# Autodesk Inventor assembly: MainModule
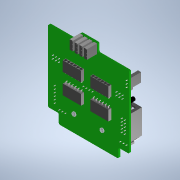
[picture p0: Inventor's stored thumbnail of the model, 180x180]
Saved by Autodesk Inventor 2021 (Build 250183000, 183)
## iProperties
Created: 2021-05-14
Part Number: MainModule
Document SubType Name: Assembly
Designer: ermoz
Author: ermoz
## Documents named in this file (19)
- D:\Moje Wyczyny\My_Poor_Projects\Sneak100_MiniSumo\minisumo-sneak100\mechanics\ElectricElements\MainModule.iam
- D:\Moje Wyczyny\My_Poor_Projects\Sneak100_MiniSumo\minisumo-sneak100\mechanics\ElectricElements\MainBoard.ipt
- D:\Moje Wyczyny\My_Poor_Projects\Sneak100_MiniSumo\minisumo-sneak100\mechanics\ElectricElements\IDC_10_pin_connector.ipt
- D:\Moje Wyczyny\My_Poor_Projects\Sneak100_MiniSumo\minisumo-sneak100\mechanics\ElectricElements\STM32F303RE_LQFP64.ipt
- D:\Moje Wyczyny\My_Poor_Projects\Sneak100_MiniSumo\minisumo-sneak100\mechanics\ElectricElements\SSD1306.ipt
- D:\Moje Wyczyny\My_Poor_Projects\Sneak100_MiniSumo\minisumo-sneak100\mechanics\ElectricElements\TactSwitch_6x6_8mm_SMD.ipt
- D:\Moje Wyczyny\My_Poor_Projects\Sneak100_MiniSumo\minisumo-sneak100\mechanics\ElectricElements\FemaleHeaderPin_1x6.iam
- D:\Moje Wyczyny\My_Poor_Projects\Sneak100_MiniSumo\minisumo-sneak100\mechanics\ElectricElements\Switch_ESP2010_90.ipt
- D:\Moje Wyczyny\My_Poor_Projects\Sneak100_MiniSumo\minisumo-sneak100\mechanics\ElectricElements\S9V11F5.ipt
- D:\Moje Wyczyny\My_Poor_Projects\Sneak100_MiniSumo\minisumo-sneak100\mechanics\ElectricElements\MaleHeaderPin_1x3.iam
- D:\Moje Wyczyny\My_Poor_Projects\Sneak100_MiniSumo\minisumo-sneak100\mechanics\ElectricElements\MaleHeaderPin_1x4.iam
- D:\Moje Wyczyny\My_Poor_Projects\Sneak100_MiniSumo\minisumo-sneak100\mechanics\ElectricElements\TSOP4838.ipt
- D:\Moje Wyczyny\My_Poor_Projects\Sneak100_MiniSumo\minisumo-sneak100\mechanics\ElectricElements\FemaleHeaderPin_1x3.iam
- D:\Moje Wyczyny\My_Poor_Projects\Sneak100_MiniSumo\minisumo-sneak100\mechanics\ElectricElements\FemaleHeaderPin_1x6_90.iam
- D:\Moje Wyczyny\My_Poor_Projects\Sneak100_MiniSumo\minisumo-sneak100\mechanics\PreMadeParts\DistanceRing_4mm.ipt
- D:\Moje Wyczyny\My_Poor_Projects\Sneak100_MiniSumo\minisumo-sneak100\mechanics\PreMadeParts\M2_Short_Bolt.ipt
- D:\Moje Wyczyny\My_Poor_Projects\Sneak100_MiniSumo\minisumo-sneak100\mechanics\ElectricElements\FemaleHeaderPin_2x3_90.iam
- D:\Moje Wyczyny\My_Poor_Projects\Sneak100_MiniSumo\minisumo-sneak100\mechanics\ElectricElements\PinHeaderJumper.ipt
- D:\Moje Wyczyny\My_Poor_Projects\Sneak100_MiniSumo\minisumo-sneak100\mechanics\PreMadeParts\2M_Nut.ipt
## Components (33 placed, 18 different names)
1. MainBoard:1 — Mate:1, Mate:3, Flush:1, Mate:8, Mate:17, Mate:18, Mate:19, Mate:24, Flush:4, Mate:25, Mate:27, Mate:32, Mate:34, Flush:11, Flush:13, Flush:14, Mate:39, Flush:15, Mate:40, Flush:16, Mate:42, Flush:17, Mate:43, Mate:44, Mate:45, Mate:46, Flush:18, Flush:19, Flush:20, Flush:21, Flush:22, Flush:23, Mate:49, Flush:24, Flush:25, Mate:50, Mate:51, Mate:52, Mate:53, Flush:30, Flush:31, Mate:55, Mate:56, Mate:57, Mate:58, Mate:59, Mate:60, Tangent:4, Tangent:5, Tangent:6, Tangent:7, Mate:63, Mate:64, Flush:33, Flush:34, Flush:35
2. IDC_10_pin_connector:1 — Mate:1, Flush:1, Flush:11, Mate:41, Mate:66
3. STM32F303RE_LQFP64:1 — Mate:3
4. SSD1306:1 — Mate:8, Tangent:1, Tangent:2, Tangent:3, Mate:36, Mate:37, Angle:4, Mate:69, Mate:70
5. TactSwitch_6x6_8mm_SMD:1 — Mate:17, Symmetry:1, Flush:2
6. TactSwitch_6x6_8mm_SMD:2 — Mate:18, Mate:20, Angle:3, Flush:2, Flush:3, Mate:35
7. TactSwitch_6x6_8mm_SMD:3 — Mate:19, Symmetry:1, Flush:3, Mate:34, Mate:35, Mate:36
8. FemaleHeaderPin_1x6:1 [sub-assembly] — Mate:24, Flush:13, Flush:14
9. Switch_ESP2010_90:1 — Flush:4, Mate:25, Flush:15
10. S9V11F5:1 — Mate:28, Flush:6, Flush:7
11. MaleHeaderPin_1x3:1 [sub-assembly] — Mate:27, Mate:28, Flush:6, Flush:7
12. MaleHeaderPin_1x4:1 [sub-assembly] — Mate:32, Tangent:1, Tangent:2, Tangent:3
13. TSOP4838:1 — Mate:39
14. TactSwitch_6x6_8mm_SMD:4 — Mate:40, Flush:16, Mate:41
15. MaleHeaderPin_1x3:2 [sub-assembly] — Mate:42, Flush:17, Mate:65, Flush:36, Flush:37, Mate:66
16. FemaleHeaderPin_1x3:1 [sub-assembly] — Mate:43, Flush:18, Flush:23, Mate:48
17. FemaleHeaderPin_1x3:2 [sub-assembly] — Mate:44, Flush:19, Mate:48
18. FemaleHeaderPin_1x3:3 [sub-assembly] — Mate:45, Flush:20, Mate:47
19. FemaleHeaderPin_1x3:4 [sub-assembly] — Mate:46, Flush:21, Flush:22, Mate:47
20. FemaleHeaderPin_1x3:5 [sub-assembly] — Mate:49, Flush:24, Flush:25
21. FemaleHeaderPin_1x6_90:1 [sub-assembly] — Mate:50, Flush:27, Flush:29
22. FemaleHeaderPin_1x6_90:2 [sub-assembly] — Mate:52, Flush:27, Flush:28, Mate:56
23. FemaleHeaderPin_1x6_90:3 [sub-assembly] — Mate:51, Flush:26, Flush:29, Flush:30
24. FemaleHeaderPin_1x6_90:4 [sub-assembly] — Mate:53, Flush:26, Flush:28, Flush:31, Mate:55
25. DistanceRing_4mm:1 — Mate:57, Mate:62
26. DistanceRing_4mm:2 — Mate:58, Mate:61
27. M2_Short_Bolt:1 — Mate:59, Mate:61, Tangent:4, Tangent:6, Mate:67
28. M2_Short_Bolt:2 — Mate:60, Mate:62, Tangent:5, Tangent:7, Mate:68
29. FemaleHeaderPin_2x3_90:1 [sub-assembly] — Mate:63, Flush:32, Flush:33
30. FemaleHeaderPin_2x3_90:2 [sub-assembly] — Mate:64, Flush:32, Flush:34, Flush:35
31. PinHeaderJumper:1 — Mate:65, Flush:36, Flush:37
32. 2M_Nut:1 — Mate:67, Mate:69
33. 2M_Nut:2 — Mate:68, Mate:70
## Relationships (93: Mate 51, Flush 32, Tangent 7, Angle 2, Symmetry 1)
- Mate:1: MainBoard:1 ↔ IDC_10_pin_connector:1
- Mate:3: MainBoard:1 ↔ STM32F303RE_LQFP64:1
- Flush:1: MainBoard:1 ↔ IDC_10_pin_connector:1
- Mate:8 (4 mm): MainBoard:1 ↔ SSD1306:1
- Mate:16
- Mate:17: MainBoard:1 ↔ TactSwitch_6x6_8mm_SMD:1
- Mate:18: MainBoard:1 ↔ TactSwitch_6x6_8mm_SMD:2
- Mate:19: MainBoard:1 ↔ TactSwitch_6x6_8mm_SMD:3
- Mate:20: TactSwitch_6x6_8mm_SMD:2
- Angle:3 (0 deg): TactSwitch_6x6_8mm_SMD:2
- Symmetry:1: TactSwitch_6x6_8mm_SMD:1 ↔ TactSwitch_6x6_8mm_SMD:3
- Mate:21
- Flush:2: TactSwitch_6x6_8mm_SMD:1 ↔ TactSwitch_6x6_8mm_SMD:2
- Flush:3: TactSwitch_6x6_8mm_SMD:2 ↔ TactSwitch_6x6_8mm_SMD:3
- Mate:23
- Mate:24: MainBoard:1 ↔ FemaleHeaderPin_1x6:1
- Flush:4 (1 mm): MainBoard:1 ↔ Switch_ESP2010_90:1
- Mate:25: MainBoard:1 ↔ Switch_ESP2010_90:1
- Mate:27: MainBoard:1 ↔ MaleHeaderPin_1x3:1
- Mate:28: S9V11F5:1 ↔ MaleHeaderPin_1x3:1
- Flush:6: S9V11F5:1 ↔ MaleHeaderPin_1x3:1
- Flush:7: S9V11F5:1 ↔ MaleHeaderPin_1x3:1
- Mate:32: MainBoard:1 ↔ MaleHeaderPin_1x4:1
- Tangent:1 (-0.225 mm): SSD1306:1 ↔ MaleHeaderPin_1x4:1
- Tangent:2 (-0.225 mm): SSD1306:1 ↔ MaleHeaderPin_1x4:1
- Mate:34 (-7 mm): MainBoard:1 ↔ TactSwitch_6x6_8mm_SMD:3
- Tangent:3 (-0.225 mm): SSD1306:1 ↔ MaleHeaderPin_1x4:1
- Mate:35 (7 mm): TactSwitch_6x6_8mm_SMD:2 ↔ TactSwitch_6x6_8mm_SMD:3
- Flush:11 (16 mm): MainBoard:1 ↔ IDC_10_pin_connector:1
- Flush:13 (13 mm): MainBoard:1 ↔ FemaleHeaderPin_1x6:1
- Flush:14 (5 mm): MainBoard:1 ↔ FemaleHeaderPin_1x6:1
- Mate:36 (9.5 mm): SSD1306:1 ↔ TactSwitch_6x6_8mm_SMD:3
- Mate:37: SSD1306:1
- Angle:4 (0 deg): SSD1306:1
- Mate:38
- Mate:39 (3 mm): MainBoard:1 ↔ TSOP4838:1
- Flush:15: MainBoard:1 ↔ Switch_ESP2010_90:1
- Mate:40: MainBoard:1 ↔ TactSwitch_6x6_8mm_SMD:4
- Flush:16 (2.77 mm): MainBoard:1 ↔ TactSwitch_6x6_8mm_SMD:4
- Mate:41 (0.9 mm): IDC_10_pin_connector:1 ↔ TactSwitch_6x6_8mm_SMD:4
- Mate:42: MainBoard:1 ↔ MaleHeaderPin_1x3:2
- Flush:17 (12.5 mm): MainBoard:1 ↔ MaleHeaderPin_1x3:2
- Mate:43: MainBoard:1 ↔ FemaleHeaderPin_1x3:1
- Mate:44: MainBoard:1 ↔ FemaleHeaderPin_1x3:2
- Mate:45: MainBoard:1 ↔ FemaleHeaderPin_1x3:3
- Mate:46: MainBoard:1 ↔ FemaleHeaderPin_1x3:4
- Flush:18 (0.2 mm): MainBoard:1 ↔ FemaleHeaderPin_1x3:1
- Flush:19 (0.4 mm): MainBoard:1 ↔ FemaleHeaderPin_1x3:2
- Flush:20 (0.4 mm): MainBoard:1 ↔ FemaleHeaderPin_1x3:3
- Flush:21 (0.4 mm): MainBoard:1 ↔ FemaleHeaderPin_1x3:4
- Flush:22 (0.4 mm): MainBoard:1 ↔ FemaleHeaderPin_1x3:4
- Flush:23 (0.2 mm): MainBoard:1 ↔ FemaleHeaderPin_1x3:1
- Mate:47 (1.4 mm): FemaleHeaderPin_1x3:3 ↔ FemaleHeaderPin_1x3:4
- Mate:48 (1.5 mm): FemaleHeaderPin_1x3:1 ↔ FemaleHeaderPin_1x3:2
- Mate:49: MainBoard:1 ↔ FemaleHeaderPin_1x3:5
- Flush:24 (0.2 mm): MainBoard:1 ↔ FemaleHeaderPin_1x3:5
- Flush:25 (5.84 mm): MainBoard:1 ↔ FemaleHeaderPin_1x3:5
- Mate:50: MainBoard:1 ↔ FemaleHeaderPin_1x6_90:1
- Mate:51: MainBoard:1 ↔ FemaleHeaderPin_1x6_90:3
- Mate:52: MainBoard:1 ↔ FemaleHeaderPin_1x6_90:2
- Mate:53: MainBoard:1 ↔ FemaleHeaderPin_1x6_90:4
- Flush:26: FemaleHeaderPin_1x6_90:3 ↔ FemaleHeaderPin_1x6_90:4
- Flush:27: FemaleHeaderPin_1x6_90:1 ↔ FemaleHeaderPin_1x6_90:2
- Flush:28: FemaleHeaderPin_1x6_90:2 ↔ FemaleHeaderPin_1x6_90:4
- Flush:29: FemaleHeaderPin_1x6_90:1 ↔ FemaleHeaderPin_1x6_90:3
- Flush:30 (14.92 mm): MainBoard:1 ↔ FemaleHeaderPin_1x6_90:3
- Flush:31 (14.92 mm): MainBoard:1 ↔ FemaleHeaderPin_1x6_90:4
- Mate:55 (-33.74 mm): MainBoard:1 ↔ FemaleHeaderPin_1x6_90:4
- Mate:56 (-32.84 mm): MainBoard:1 ↔ FemaleHeaderPin_1x6_90:2
- Mate:57: MainBoard:1 ↔ DistanceRing_4mm:1
- Mate:58: MainBoard:1 ↔ DistanceRing_4mm:2
- Mate:59: MainBoard:1 ↔ M2_Short_Bolt:1
- Mate:60: MainBoard:1 ↔ M2_Short_Bolt:2
- Mate:61: DistanceRing_4mm:2 ↔ M2_Short_Bolt:1
- Mate:62: DistanceRing_4mm:1 ↔ M2_Short_Bolt:2
- Tangent:4 (-15.25 mm): MainBoard:1 ↔ M2_Short_Bolt:1
- Tangent:5 (-15.25 mm): MainBoard:1 ↔ M2_Short_Bolt:2
- Tangent:6 (-23.25 mm): MainBoard:1 ↔ M2_Short_Bolt:1
- Tangent:7 (-23.25 mm): MainBoard:1 ↔ M2_Short_Bolt:2
- Mate:63: MainBoard:1 ↔ FemaleHeaderPin_2x3_90:1
- Mate:64: MainBoard:1 ↔ FemaleHeaderPin_2x3_90:2
- Flush:32: FemaleHeaderPin_2x3_90:1 ↔ FemaleHeaderPin_2x3_90:2
- Flush:33 (3.6 mm): MainBoard:1 ↔ FemaleHeaderPin_2x3_90:1
- Flush:34 (3.6 mm): MainBoard:1 ↔ FemaleHeaderPin_2x3_90:2
- Flush:35 (9.87 mm): MainBoard:1 ↔ FemaleHeaderPin_2x3_90:2
- Mate:65: MaleHeaderPin_1x3:2 ↔ PinHeaderJumper:1
- Flush:36: MaleHeaderPin_1x3:2 ↔ PinHeaderJumper:1
- Flush:37: MaleHeaderPin_1x3:2 ↔ PinHeaderJumper:1
- Mate:66 (0.87 mm): IDC_10_pin_connector:1 ↔ MaleHeaderPin_1x3:2
- Mate:67: M2_Short_Bolt:1 ↔ 2M_Nut:1
- Mate:68: M2_Short_Bolt:2 ↔ 2M_Nut:2
- Mate:69: SSD1306:1 ↔ 2M_Nut:1
- Mate:70: SSD1306:1 ↔ 2M_Nut:2
